# Autodesk Inventor assembly: VER2.0_MIR_CPY
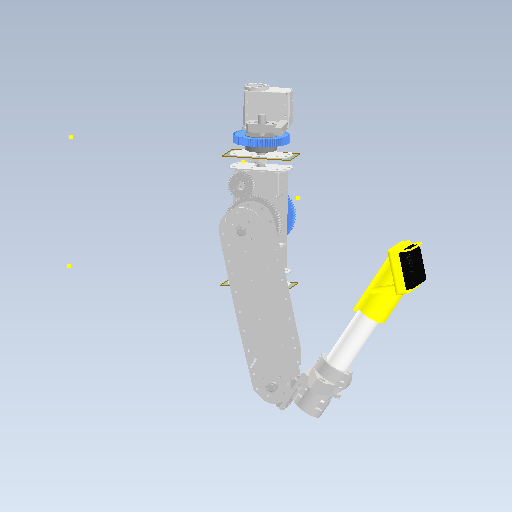
[picture p0: Inventor's stored thumbnail of the model, 512x512]
Saved by Autodesk Inventor 2020 (Build 240168000, 168)
## iProperties
Created: 2022-10-31
Part Number: VER2.0_MIR_CPY
Document SubType Name: Assembly
Designer: kanazawakotaro
Author: Administrator
## Documents named in this file (26)
- C:\Users\satolab\Documents\kamuy2\VER2.0_MIR_CPY.iam
- C:\Users\satolab\Documents\kamuy2\Parts\Part2_MIR_CPY.ipt
- C:\Users\satolab\Documents\kamuy2\Parts\x-540_idle_MIR_CPY.ipt
- C:\Users\satolab\Documents\kamuy2\Parts\GEABP1.0-32-10-A-12-KFC22-K3_Autodesk_Inventor_2020_20221101\AIS2020\GEABP1_0-32-10-A-12-KFC22-K3_MIR_CPY.iam
- C:\Users\satolab\Documents\kamuy2\Parts\GEYK1.0-70-10-B-10K_Autodesk_Inventor_2020_20221114\AIS2020\GEYK1_0-70-10-B-10K_MIR_CPY.iam
- C:\Users\satolab\Documents\kamuy2\Part16_MIR_CPY.ipt
- C:\Users\satolab\Documents\kamuy2\Part1_MIR_CPY.ipt
- C:\Users\satolab\Documents\kamuy2\Part13_MIR_CPY.ipt
- C:\Users\satolab\Documents\kamuy2\Part17_MIR_CPY.ipt
- C:\Users\satolab\Documents\kamuy2\Parts\SMYHF10_STEP_AP203AP214\SMYHF10_203_MIR_CPY.ipt
- C:\Users\satolab\Documents\kamuy2\Parts\BGHK6800VV-30_Autodesk_Inventor_2020_20221102\AIS2020\BGHK6800VV-30_MIR_CPY.iam
- C:\Users\satolab\Documents\kamuy2\Parts\XW540.N105.I101_MIR_CPY.ipt
- C:\Users\satolab\Documents\kamuy2\Parts\NSFMKR10-67-KA22-A20_Autodesk_Inventor_2020_20221116\AIS2020\NSFMKR10-67-KA22-A20_MIR_CPY.iam
- C:\Users\satolab\Documents\kamuy2\Parts\NSFMR10-37_Autodesk_Inventor_2020_20221116\AIS2020\NSFMR10-37(000_000)_MIR_CPY.iam
- C:\Users\satolab\Documents\kamuy2\Parts\NSFMKRRA10-144-F3-S6-KA5-A18-KB108.5-B11_Autodesk_Inventor_2020_20221117\AIS2020\NSFMKRRA10-144-F3-S6-KA5-A18-KB108_5-B11_MIR_CPY.iam
- C:\Users\satolab\Documents\kamuy2\Parts\BGTAB6900VV_Autodesk_Inventor_2020_20221121\AIS2020\BGTAB6900VV.iam
- C:\Users\satolab\Documents\kamuy2\Parts\GEABP1.0-70-10-A-19-KFC30-K3_Autodesk_Inventor_2020_20221114\AIS2020\GEABP1_0-70-10-A-19-KFC30-K3_MIR_MIR_MIR1_MIR_MIR.iam
- C:\Users\satolab\Documents\kamuy2\Parts\PIJX30-20-150_Autodesk_Inventor_2020_20221115\PIJX30-20-150_MIR_MIR_MIR1_MIR_MIR.ipt
- C:\Users\satolab\Documents\kamuy2\Parts\C-SHA10_Autodesk_Inventor_2020_20221104\AIS2020\C-SHA10_MIR_MIR_MIR1_MIR_MIR.iam
- C:\Users\satolab\Documents\kamuy2\Parts\HTPA30S3M060-A-N10_Autodesk_Inventor_2020_20221115\AIS2020\HTPA30S3M060-A-N10_MIR_MIR_MIR1_MIR_MIR.iam
- C:\Users\satolab\Documents\kamuy2\Part20_MIR_MIR_MIR1_MIR_MIR.ipt
- C:\Users\satolab\Documents\kamuy2\Parts\SMYHF30_STEP_AP203AP214\SMYHF30_203_MIR_MIR_MIR1_MIR_MIR.ipt
- C:\Users\satolab\Documents\kamuy2\3dprinter\Part77_MIR.ipt
- C:\Users\satolab\Documents\kamuy2\Parts\NSFMRRA10-74-B3-S3-KC31.5-A11_Autodesk_Inventor_2020_20221116\AIS2020\NSFMRRA10-74-B3-S3-KC31_5-A11(000_000)_MIR_MIR_MIR1_MIR_MIR.iam
- C:\Users\satolab\Documents\kamuy2\Parts\foot3d.ipt
- C:\Users\satolab\Documents\kamuy2\Parts\gom.ipt
## Components (39 placed, 26 different names)
1. Part2_MIR_CPY:1
2. x-540_idle_MIR_CPY:1 — メイト:50, メイト:51, フラッシュ:58, フラッシュ:66, フラッシュ:68, メイト:166, フラッシュ:103, メイト:256, メイト:102
3. GEABP1_0-32-10-A-12-KFC22-K3_MIR_CPY:1 [sub-assembly] — メイト:50, メイト:51, フラッシュ:47
4. GEYK1_0-70-10-B-10K_MIR_CPY:1 [sub-assembly] — フラッシュ:61, メイト:248, フラッシュ:136
5. x-540_idle_MIR_CPY:2 — フラッシュ:58, フラッシュ:66, フラッシュ:68, メイト:85, メイト:86, フラッシュ:100, メイト:183, メイト:178, メイト:179, メイト:180
6. GEABP1_0-32-10-A-12-KFC22-K3_MIR_CPY:2 [sub-assembly] — メイト:85, メイト:86, フラッシュ:61
7. Part16_MIR_CPY:2 — メイト:111, メイト:112, フラッシュ:50
8. Part16_MIR_CPY:3 — メイト:66, メイト:67, フラッシュ:50
9. Part1_MIR_CPY:1 — フラッシュ:100, メイト:66
10. Part1_MIR_CPY:2 — メイト:166, メイト:183, メイト:101, メイト:102, メイト:112
11. Part13_MIR_CPY:1 — フラッシュ:103, メイト:172, フラッシュ:104, フラッシュ:108, メイト:208
12. Part17_MIR_CPY:1 — メイト:172, フラッシュ:104, フラッシュ:108, メイト:174, フラッシュ:105, メイト:177
13. SMYHF10_203_MIR_CPY:1 — メイト:174, フラッシュ:105, メイト:254
14. GEYK1_0-70-10-B-10K_MIR_CPY:2 [sub-assembly] — メイト:177, メイト:207, メイト:65, メイト:71
15. Part13_MIR_CPY:2 — メイト:178, メイト:179, メイト:180, メイト:194, フラッシュ:110, メイト:214
16. SMYHF10_203_MIR_CPY:2 — メイト:185, メイト:187, メイト:213
17. Part17_MIR_CPY:2 — メイト:185, メイト:187, メイト:194, フラッシュ:110, メイト:211, メイト:215, メイト:69
18. BGHK6800VV-30_MIR_CPY:1 [sub-assembly] — メイト:205, メイト:209, フラッシュ:115, フラッシュ:116, フラッシュ:33, メイト:65, フラッシュ:34
19. GEABP1_0-32-10-A-12-KFC22-K3_MIR_CPY:3 [sub-assembly] — メイト:203, メイト:204
20. XW540.N105.I101_MIR_CPY:1 — メイト:203, メイト:204, メイト:205, フラッシュ:33, フラッシュ:34, メイト:72
21. NSFMKR10-67-KA22-A20_MIR_CPY:1 [sub-assembly] — メイト:207, メイト:208, メイト:209, メイト:254, メイト:70
22. BGHK6800VV-30_MIR_CPY:2 [sub-assembly] — フラッシュ:115, フラッシュ:116, メイト:211, メイト:212
23. NSFMR10-37(000_000)_MIR_CPY:1 [sub-assembly] — メイト:212, メイト:213, メイト:214, メイト:215, メイト:68
24. NSFMKRRA10-144-F3-S6-KA5-A18-KB108_5-B11_MIR_CPY:1 [sub-assembly] — メイト:248, フラッシュ:136, メイト:256, メイト:67, メイト:101, メイト:103, メイト:104, メイト:106, メイト:111
25. BGTAB6900VV:1 [sub-assembly] — メイト:68, メイト:69, フラッシュ:35
26. c:2 [sub-assembly] — メイト:70, メイト:71, メイト:72, フラッシュ:35
27. GEABP1_0-70-10-A-19-KFC30-K3_MIR_MIR_MIR1_MIR_MIR:2 [sub-assembly] — メイト:103, フラッシュ:47, メイト:105
28. PIJX30-20-150_MIR_MIR_MIR1_MIR_MIR:2 — メイト:109, メイト:110
29. C-SHA10_MIR_MIR_MIR1_MIR_MIR:3 [sub-assembly]
30. C-SHA10_MIR_MIR_MIR1_MIR_MIR:4 [sub-assembly]
31. HTPA30S3M060-A-N10_MIR_MIR_MIR1_MIR_MIR:3 [sub-assembly]
32. HTPA30S3M060-A-N10_MIR_MIR_MIR1_MIR_MIR:4 [sub-assembly]
33. Part20_MIR_MIR_MIR1_MIR_MIR:3 — メイト:105
34. SMYHF30_203_MIR_MIR_MIR1_MIR_MIR:2
35. NSFMRRA10-74-B3-S3-KC31_5-A11(000_000)_MIR_MIR_MIR1_MIR_MIR:1 [sub-assembly]
36. Part77_MIR:2 — フラッシュ:49
37. Part20_MIR_MIR_MIR1_MIR_MIR:4 — メイト:104, メイト:106
38. foot3d:1 — メイト:109, メイト:110, フラッシュ:49
39. gom:1
## Relationships (90: Mate 66, Flush 24)
- メイト:50 [Mate] (4 mm): x-540_idle_MIR_CPY:1 ↔ GEABP1_0-32-10-A-12-KFC22-K3_MIR_CPY:1
- メイト:51 [Mate]: x-540_idle_MIR_CPY:1 ↔ GEABP1_0-32-10-A-12-KFC22-K3_MIR_CPY:1
- フラッシュ:58 [Flush]: x-540_idle_MIR_CPY:1 ↔ x-540_idle_MIR_CPY:2
- フラッシュ:66 [Flush]: x-540_idle_MIR_CPY:1 ↔ x-540_idle_MIR_CPY:2
- フラッシュ:68 [Flush]: x-540_idle_MIR_CPY:1 ↔ x-540_idle_MIR_CPY:2
- メイト:85 [Mate]: x-540_idle_MIR_CPY:2 ↔ GEABP1_0-32-10-A-12-KFC22-K3_MIR_CPY:2
- メイト:86 [Mate] (4 mm): x-540_idle_MIR_CPY:2 ↔ GEABP1_0-32-10-A-12-KFC22-K3_MIR_CPY:2
- フラッシュ:61 [Flush]: GEYK1_0-70-10-B-10K_MIR_CPY:1 ↔ GEABP1_0-32-10-A-12-KFC22-K3_MIR_CPY:2
- フラッシュ:100 [Mate]: x-540_idle_MIR_CPY:2 ↔ Part1_MIR_CPY:1
- メイト:166 [Mate]: x-540_idle_MIR_CPY:1 ↔ Part1_MIR_CPY:2
- メイト:183 [Mate]: x-540_idle_MIR_CPY:2 ↔ Part1_MIR_CPY:2
- フラッシュ:103 [Mate]: x-540_idle_MIR_CPY:1 ↔ Part13_MIR_CPY:1
- メイト:172 [Mate] (15 mm): Part13_MIR_CPY:1 ↔ Part17_MIR_CPY:1
- フラッシュ:104 [Flush]: Part13_MIR_CPY:1 ↔ Part17_MIR_CPY:1
- フラッシュ:108 [Flush]: Part13_MIR_CPY:1 ↔ Part17_MIR_CPY:1
- メイト:174 [Mate]: Part17_MIR_CPY:1 ↔ SMYHF10_203_MIR_CPY:1
- フラッシュ:105 [Flush] (0.1 mm): Part17_MIR_CPY:1 ↔ SMYHF10_203_MIR_CPY:1
- メイト:177 [Mate] (5 mm): Part17_MIR_CPY:1 ↔ GEYK1_0-70-10-B-10K_MIR_CPY:2
- メイト:178 [Mate]: x-540_idle_MIR_CPY:2 ↔ Part13_MIR_CPY:2
- メイト:179 [Mate]: x-540_idle_MIR_CPY:2 ↔ Part13_MIR_CPY:2
- メイト:180 [Mate]: x-540_idle_MIR_CPY:2 ↔ Part13_MIR_CPY:2
- メイト:185 [Mate]: SMYHF10_203_MIR_CPY:2 ↔ Part17_MIR_CPY:2
- メイト:187 [Mate]: SMYHF10_203_MIR_CPY:2 ↔ Part17_MIR_CPY:2
- メイト:194 [Mate] (15 mm): Part13_MIR_CPY:2 ↔ Part17_MIR_CPY:2
- フラッシュ:110 [Flush]: Part13_MIR_CPY:2 ↔ Part17_MIR_CPY:2
- メイト:203 [Mate]: GEABP1_0-32-10-A-12-KFC22-K3_MIR_CPY:3 ↔ XW540.N105.I101_MIR_CPY:1
- メイト:204 [Mate]: GEABP1_0-32-10-A-12-KFC22-K3_MIR_CPY:3 ↔ XW540.N105.I101_MIR_CPY:1
- メイト:205 [Mate] (6.591 mm): BGHK6800VV-30_MIR_CPY:1 ↔ XW540.N105.I101_MIR_CPY:1
- メイト:207 [Mate]: GEYK1_0-70-10-B-10K_MIR_CPY:2 ↔ NSFMKR10-67-KA22-A20_MIR_CPY:1
- メイト:208 [Mate]: Part13_MIR_CPY:1 ↔ NSFMKR10-67-KA22-A20_MIR_CPY:1
- メイト:209 [Mate]: BGHK6800VV-30_MIR_CPY:1 ↔ NSFMKR10-67-KA22-A20_MIR_CPY:1
- メイト:254 [Mate]: SMYHF10_203_MIR_CPY:1 ↔ NSFMKR10-67-KA22-A20_MIR_CPY:1
- フラッシュ:115 [Flush]: BGHK6800VV-30_MIR_CPY:1 ↔ BGHK6800VV-30_MIR_CPY:2
- フラッシュ:116 [Flush]: BGHK6800VV-30_MIR_CPY:1 ↔ BGHK6800VV-30_MIR_CPY:2
- メイト:211 [Mate] (4 mm): Part17_MIR_CPY:2 ↔ BGHK6800VV-30_MIR_CPY:2
- メイト:212 [Mate]: BGHK6800VV-30_MIR_CPY:2 ↔ NSFMR10-37(000_000)_MIR_CPY:1
- メイト:213 [Mate]: SMYHF10_203_MIR_CPY:2 ↔ NSFMR10-37(000_000)_MIR_CPY:1
- メイト:214 [Mate]: Part13_MIR_CPY:2 ↔ NSFMR10-37(000_000)_MIR_CPY:1
- メイト:215 [Mate]: Part17_MIR_CPY:2 ↔ NSFMR10-37(000_000)_MIR_CPY:1
- メイト:248 [Mate]: GEYK1_0-70-10-B-10K_MIR_CPY:1 ↔ NSFMKRRA10-144-F3-S6-KA5-A18-KB108_5-B11_MIR_CPY:1
- フラッシュ:136 [Flush] (-3 mm): GEYK1_0-70-10-B-10K_MIR_CPY:1 ↔ NSFMKRRA10-144-F3-S6-KA5-A18-KB108_5-B11_MIR_CPY:1
- メイト:256 [Mate] (31.591 mm): x-540_idle_MIR_CPY:1 ↔ NSFMKRRA10-144-F3-S6-KA5-A18-KB108_5-B11_MIR_CPY:1
- フラッシュ:33 [Flush]: BGHK6800VV-30_MIR_CPY:1 ↔ XW540.N105.I101_MIR_CPY:1
- メイト:65 [Mate] (4 mm): GEYK1_0-70-10-B-10K_MIR_CPY:2 ↔ BGHK6800VV-30_MIR_CPY:1
- フラッシュ:34 [Flush]: BGHK6800VV-30_MIR_CPY:1 ↔ XW540.N105.I101_MIR_CPY:1
- メイト:66 [Mate]: Part16_MIR_CPY:3 ↔ Part1_MIR_CPY:1
- メイト:67 [Mate]: Part16_MIR_CPY:3 ↔ NSFMKRRA10-144-F3-S6-KA5-A18-KB108_5-B11_MIR_CPY:1
- メイト:68 [Mate]: NSFMR10-37(000_000)_MIR_CPY:1 ↔ BGTAB6900VV:1
- メイト:69 [Mate] (4 mm): Part17_MIR_CPY:2 ↔ BGTAB6900VV:1
- メイト:70 [Mate]: NSFMKR10-67-KA22-A20_MIR_CPY:1 ↔ c:2
- メイト:71 [Mate] (4 mm): GEYK1_0-70-10-B-10K_MIR_CPY:2 ↔ c:2
- メイト:72 [Mate] (18.591 mm): XW540.N105.I101_MIR_CPY:1 ↔ c:2
- フラッシュ:35 [Flush]: BGTAB6900VV:1 ↔ c:2
- [Flush]: C-SHA10_MIR_MIR_MIR1_MIR_MIR:3 ↔ C-SHA10_MIR_MIR_MIR1_MIR_MIR:4
- [Flush]: C-SHA10_MIR_MIR_MIR1_MIR_MIR:3 ↔ C-SHA10_MIR_MIR_MIR1_MIR_MIR:4
- [Mate]: C-SHA10_MIR_MIR_MIR1_MIR_MIR:4 ↔ HTPA30S3M060-A-N10_MIR_MIR_MIR1_MIR_MIR:3
- [Mate]: GEABP1_0-70-10-A-19-KFC30-K3_MIR_MIR_MIR1_MIR_MIR:2 ↔ HTPA30S3M060-A-N10_MIR_MIR_MIR1_MIR_MIR:4
- [Flush]: HTPA30S3M060-A-N10_MIR_MIR_MIR1_MIR_MIR:3 ↔ HTPA30S3M060-A-N10_MIR_MIR_MIR1_MIR_MIR:4
- [Mate]: HTPA30S3M060-A-N10_MIR_MIR_MIR1_MIR_MIR:4 ↔ Part20_MIR_MIR_MIR1_MIR_MIR:3
- [Mate] (6 mm): C-SHA10_MIR_MIR_MIR1_MIR_MIR:4 ↔ Part20_MIR_MIR_MIR1_MIR_MIR:3
- [Flush] (-20 mm): PIJX30-20-150_MIR_MIR_MIR1_MIR_MIR:2 ↔ SMYHF30_203_MIR_MIR_MIR1_MIR_MIR:2
- [Flush] (-20 mm): C-SHA10_MIR_MIR_MIR1_MIR_MIR:4 ↔ SMYHF30_203_MIR_MIR_MIR1_MIR_MIR:2
- [Mate] (15 mm): C-SHA10_MIR_MIR_MIR1_MIR_MIR:4 ↔ SMYHF30_203_MIR_MIR_MIR1_MIR_MIR:2
- [Mate]: PIJX30-20-150_MIR_MIR_MIR1_MIR_MIR:2 ↔ SMYHF30_203_MIR_MIR_MIR1_MIR_MIR:2
- [Flush] (31.5 mm): HTPA30S3M060-A-N10_MIR_MIR_MIR1_MIR_MIR:3 ↔ NSFMRRA10-74-B3-S3-KC31_5-A11(000_000)_MIR_MIR_MIR1_MIR_MIR:1
- [Mate]: C-SHA10_MIR_MIR_MIR1_MIR_MIR:3 ↔ NSFMRRA10-74-B3-S3-KC31_5-A11(000_000)_MIR_MIR_MIR1_MIR_MIR:1
- [Mate]: HTPA30S3M060-A-N10_MIR_MIR_MIR1_MIR_MIR:3 ↔ NSFMRRA10-74-B3-S3-KC31_5-A11(000_000)_MIR_MIR_MIR1_MIR_MIR:1
- [Mate]: Part20_MIR_MIR_MIR1_MIR_MIR:3 ↔ NSFMRRA10-74-B3-S3-KC31_5-A11(000_000)_MIR_MIR_MIR1_MIR_MIR:1
- [Mate]: Part20_MIR_MIR_MIR1_MIR_MIR:3 ↔ NSFMRRA10-74-B3-S3-KC31_5-A11(000_000)_MIR_MIR_MIR1_MIR_MIR:1
- [Mate]: SMYHF30_203_MIR_MIR_MIR1_MIR_MIR:2 ↔ Part77_MIR:2
- [Mate]: PIJX30-20-150_MIR_MIR_MIR1_MIR_MIR:2 ↔ Part77_MIR:2
- [Mate]: C-SHA10_MIR_MIR_MIR1_MIR_MIR:4 ↔ Part77_MIR:2
- [Mate]: C-SHA10_MIR_MIR_MIR1_MIR_MIR:3 ↔ HTPA30S3M060-A-N10_MIR_MIR_MIR1_MIR_MIR:3
- [Mate]: NSFMRRA10-74-B3-S3-KC31_5-A11(000_000)_MIR_MIR_MIR1_MIR_MIR:1 ↔ Part20_MIR_MIR_MIR1_MIR_MIR:4
- メイト:101 [Mate]: Part1_MIR_CPY:2 ↔ NSFMKRRA10-144-F3-S6-KA5-A18-KB108_5-B11_MIR_CPY:1
- メイト:102 [Mate]: x-540_idle_MIR_CPY:1 ↔ Part1_MIR_CPY:2
- メイト:103 [Mate]: NSFMKRRA10-144-F3-S6-KA5-A18-KB108_5-B11_MIR_CPY:1 ↔ GEABP1_0-70-10-A-19-KFC30-K3_MIR_MIR_MIR1_MIR_MIR:2
- フラッシュ:47 [Flush]: GEABP1_0-32-10-A-12-KFC22-K3_MIR_CPY:1 ↔ GEABP1_0-70-10-A-19-KFC30-K3_MIR_MIR_MIR1_MIR_MIR:2
- メイト:104 [Mate]: NSFMKRRA10-144-F3-S6-KA5-A18-KB108_5-B11_MIR_CPY:1 ↔ Part20_MIR_MIR_MIR1_MIR_MIR:4
- メイト:105 [Mate]: GEABP1_0-70-10-A-19-KFC30-K3_MIR_MIR_MIR1_MIR_MIR:2 ↔ Part20_MIR_MIR_MIR1_MIR_MIR:3
- メイト:106 [Mate]: NSFMKRRA10-144-F3-S6-KA5-A18-KB108_5-B11_MIR_CPY:1 ↔ Part20_MIR_MIR_MIR1_MIR_MIR:4
- [Flush]: foot3d:1 ↔ gom:1
- [Mate]: foot3d:1 ↔ gom:1
- [Mate]: foot3d:1 ↔ gom:1
- メイト:109 [Mate]: PIJX30-20-150_MIR_MIR_MIR1_MIR_MIR:2 ↔ foot3d:1
- メイト:110 [Mate]: PIJX30-20-150_MIR_MIR_MIR1_MIR_MIR:2 ↔ foot3d:1
- フラッシュ:49 [Flush] (10 mm): Part77_MIR:2 ↔ foot3d:1
- メイト:111 [Mate]: Part16_MIR_CPY:2 ↔ NSFMKRRA10-144-F3-S6-KA5-A18-KB108_5-B11_MIR_CPY:1
- メイト:112 [Mate]: Part16_MIR_CPY:2 ↔ Part1_MIR_CPY:2
- フラッシュ:50 [Flush]: Part16_MIR_CPY:2 ↔ Part16_MIR_CPY:3
## Named parameters: d132_d85 = 0 mm, d134_d61_d48 = 0 mm, d135_d62_d49 = 0 mm, d136_d63_d50 = 0 mm, d137_d64_d51 = 0 mm, d138_d65_d52 = 0 mm, d139_d53 = 0 mm, d140_d68_d55 = 6 mm, d142_d70_d60 = -20 mm, d143_d61 = -20 mm, d144_d62 = 15 mm, d145_d63 = 0 mm, d151_d74 = 0 mm, d152_d75 = 0 mm, d153_d76 = 0 mm
